# Autodesk Inventor assembly: Chain Testing
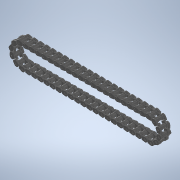
[picture p0: Inventor's stored thumbnail of the model, 180x180]
Saved by Autodesk Inventor 2020 (Build 240168000, 168)
## iProperties
Created: 2019-09-16
Part Number: Chain Testing
Document SubType Name: Assembly
Designer: Corey
Author: Corey
## Documents named in this file (3)
- C:\Users\Corey\Documents\Tower-Takeover-CAD\Chain Testing.iam
- C:\Users\Corey\Documents\Tower-Takeover-CAD\Chain Sketch.ipt
- C:\Users\Corey\Documents\Tower-Takeover-CAD\Parts\Motion\Chain & Tank Tread\Chain Link.ipt
## Components (53 placed, 2 different names)
1. Chain Sketch:1 — Mate:1, Mate:2, Flush:1
2. Chain Link:1 — Mate:1, Mate:2, Flush:1
3. Chain Link:2
4. Chain Link:3
5. Chain Link:4
6. Chain Link:5
7. Chain Link:6
8. Chain Link:7
9. Chain Link:8
10. Chain Link:9
11. Chain Link:10
12. Chain Link:11
13. Chain Link:12
14. Chain Link:13
15. Chain Link:14
16. Chain Link:15
17. Chain Link:16
18. Chain Link:17
19. Chain Link:18
20. Chain Link:19
21. Chain Link:20
22. Chain Link:21
23. Chain Link:22
24. Chain Link:23
25. Chain Link:24
26. Chain Link:25
27. Chain Link:26
28. Chain Link:27
29. Chain Link:28
30. Chain Link:29
31. Chain Link:30
32. Chain Link:31
33. Chain Link:32
34. Chain Link:33
35. Chain Link:34
36. Chain Link:35
37. Chain Link:36
38. Chain Link:37
39. Chain Link:38
40. Chain Link:39
41. Chain Link:40
42. Chain Link:41
43. Chain Link:42
44. Chain Link:43
45. Chain Link:44
46. Chain Link:45
47. Chain Link:46
48. Chain Link:47
49. Chain Link:48
50. Chain Link:49
51. Chain Link:50
52. Chain Link:51
53. Chain Link:52
## Component patterns: (52 elements, first: Chain Link:1)
## Relationships (3: Mate 2, Flush 1)
- Mate:1 (76.2 mm): Chain Sketch:1 ↔ Chain Link:1
- Mate:2: Chain Sketch:1 ↔ Chain Link:1
- Flush:1 (6.35 mm): Chain Sketch:1 ↔ Chain Link:1
